# Autodesk Inventor assembly: ASY PNS 1600 Filter column D1000
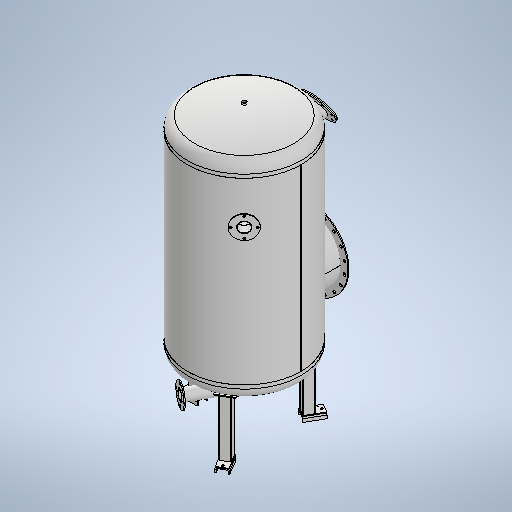
[picture p0: Inventor's stored thumbnail of the model, 512x512]
Saved by Autodesk Inventor 2025.3 (Build 293356030, 356C)
## iProperties
Created: 2025-02-13
Part Number: ASY PNS 1600 Filter column D1000
Document SubType Name: Assembly
Designer: pokla
Author: pokla
Revision Number: 3
## Documents named in this file (23)
- C:\Users\admin\Yandex.Disk\home pc\Inventor\SLM Salemal\ASY SLM 1600 Filter column D1000.iam
- C:\Users\admin\Yandex.Disk\home pc\Inventor\SLM Salemal\PNS-612 accses hatch flangeipt.ipt
- C:\Users\admin\Yandex.Disk\home pc\Inventor\SLM Salemal\PNS 1601 DIM Filter column D1000.ipt
- C:\Users\admin\Yandex.Disk\home pc\Inventor\SLM Salemal\PNS-611 accses hatch tube.ipt
- C:\Users\admin\Yandex.Disk\home pc\Inventor\SLM Salemal\PNS 1602 main Shell D1000.ipt
- C:\Users\admin\Yandex.Disk\home pc\Inventor\SLM Salemal\PNS 1604 dished head D1000.ipt
- C:\Users\admin\Yandex.Disk\home pc\Inventor\SLM Salemal\Fitting G1.ipt
- C:\Users\admin\Yandex.Disk\home pc\Inventor\SLM Salemal\ASY PNS 1690 Filter legs D1000.iam
- C:\Users\admin\Yandex.Disk\home pc\Inventor\SLM Salemal\PNS 1633 charging blind flange.ipt
- C:\Users\admin\Yandex.Disk\home pc\Inventor\SLM Salemal\ASY PNS 1610 charging hatch.iam
- C:\Users\admin\Yandex.Disk\home pc\Inventor\Content Center Files\en-US\JIS B 2312 90 (2)\JIS B 2312 90 Deg Long Elbow Steel 80A x Sch 40.ipt
- C:\Users\admin\Yandex.Disk\home pc\Inventor\SLM Salemal\ASY PNS 1650 filter-distribution-system 1000.iam
- C:\Users\admin\Yandex.Disk\home pc\Inventor\SLM Salemal\PNS 1612 FDS tube 2.ipt
- C:\Users\admin\Yandex.Disk\home pc\Inventor\SLM Salemal\PNS 1604 charging tube.ipt
- C:\Users\admin\Yandex.Disk\home pc\Inventor\SLM Salemal\PNS 1606 charging flange round.ipt
- C:\Users\admin\Yandex.Disk\home pc\Inventor\SLM Salemal\PNS 1607 charging flange cup.ipt
- C:\Users\admin\Yandex.Disk\home pc\Inventor\SLM Salemal\PNS 1613 FDS tube 3.ipt
- C:\Users\admin\Yandex.Disk\home pc\Inventor\SLM Salemal\PNS 1614 FDS tube 4.ipt
- C:\Users\admin\Yandex.Disk\home pc\Inventor\SLM Salemal\PNS 1615 FDS tube 5.ipt
- C:\Users\admin\Yandex.Disk\home pc\Inventor\SLM Salemal\ASY PNS 179 top funnel 1200 50-90_1000x90.iam
- C:\Users\admin\Yandex.Disk\home pc\Inventor\SLM Salemal\pallet jack dummy.ipt
- C:\Users\admin\Yandex.Disk\home pc\Inventor\SLM Salemal\SLM 1431 FDS flange DN90.ipt
- C:\Users\admin\Yandex.Disk\home pc\Inventor\SLM Salemal\SLM 1432 FDS free flange DN90.ipt
## Components (27 placed, 23 different names)
1. PNS 1601 DIM Filter column D1000.ipt:1
2. PNS-612 accses hatch flangeipt.ipt:1 — Rotational:73, Rotational:74
3. PNS-611 accses hatch tube.ipt:1 — Rigid:10, Rotational:74
4. PNS 1602 main Shell D1000.ipt:1 — Rigid:10, Rigid:13, Rigid:14, Mate:1, Mate:2, Rigid:66, Rigid:74
5. PNS 1604 dished head D1000.ipt:1 — Rigid:13, Rigid:75
6. PNS 1604 dished head D1000.ipt:2 — Rigid:14, Rigid:15, Mate:3
7. Fitting G1.ipt:1 — Rigid:15
8. Fitting G1.ipt:2
9. ASY PNS 1690 Filter legs D1000.iam:1 [sub-assembly] — Flush:2, Flush:3
10. ASY PNS 1610 charging hatch.iam:1 [sub-assembly] — Rotational:73
11. PNS 1633 charging blind flange.ipt:2 — Rigid:67
12. JIS B 2312 90 Deg Long Elbow Steel 80A x Sch 40.ipt:1 — Rigid:68, Rotational:70
13. JIS B 2312 90 Deg Long Elbow Steel 80A x Sch 40.ipt:2 — Rigid:62, Rigid:73
14. ASY PNS 1650 filter-distribution-system 1000.iam:1 [sub-assembly]
15. PNS 1612 FDS tube 2:3 — Rigid:62, Rigid:78
16. PNS 1604 charging tube:1 — Rigid:64, Rigid:66
17. PNS 1606 charging flange round:1 — Rigid:64, Rigid:65
18. PNS 1607 charging flange cup:1 — Rigid:65
19. PNS 1613 FDS tube 3:1 — Rigid:67, Rigid:68, Flush:3
20. PNS 1614 FDS tube 4:1 — Rotational:70, Rigid:75, Rotational:71
21. PNS 1615 FDS tube 5:1 — Rigid:73, Rigid:74, Rigid:77
22. ASY PNS 179 top funnel 1200 50-90_1000x90:1 [sub-assembly] — Rotational:72
23. pallet jack dummy:1
24. SLM 1431 FDS flange DN90:1 — Rigid:76
25. SLM 1432 FDS free flange DN90:1 — Rotational:71, Rigid:76
26. PNS 1633 charging blind flange:5 — Rigid:77
27. PNS 1633 charging blind flange:6 — Rigid:78, Rotational:72
## Relationships (26: WeldJoint 16, RevoluteJoint 5, Mate 3, Flush 2)
- Rigid:10 [WeldJoint] (66 mm): PNS-611 accses hatch tube.ipt:1 ↔ PNS 1602 main Shell D1000.ipt:1
- Rigid:13 [WeldJoint]: PNS 1602 main Shell D1000.ipt:1 ↔ PNS 1604 dished head D1000.ipt:1
- Rigid:14 [WeldJoint]: PNS 1602 main Shell D1000.ipt:1 ↔ PNS 1604 dished head D1000.ipt:2
- Rigid:15 [WeldJoint]: PNS 1604 dished head D1000.ipt:2 ↔ Fitting G1.ipt:1
- Mate:1: PNS 1602 main Shell D1000.ipt:1
- Mate:2: PNS 1602 main Shell D1000.ipt:1
- Mate:3 (2300 mm): PNS 1604 dished head D1000.ipt:2
- Flush:2: ASY PNS 1690 Filter legs D1000.iam:1
- Rigid:62 [WeldJoint]: JIS B 2312 90 Deg Long Elbow Steel 80A x Sch 40.ipt:2 ↔ PNS 1612 FDS tube 2:3
- Rigid:64 [WeldJoint]: PNS 1604 charging tube:1 ↔ PNS 1606 charging flange round:1
- Rigid:65 [WeldJoint]: PNS 1606 charging flange round:1 ↔ PNS 1607 charging flange cup:1
- Rigid:66 [WeldJoint]: PNS 1602 main Shell D1000.ipt:1 ↔ PNS 1604 charging tube:1
- Rigid:67 [WeldJoint]: PNS 1633 charging blind flange.ipt:2 ↔ PNS 1613 FDS tube 3:1
- Rigid:68 [WeldJoint]: JIS B 2312 90 Deg Long Elbow Steel 80A x Sch 40.ipt:1 ↔ PNS 1613 FDS tube 3:1
- Rotational:70 [RevoluteJoint]: JIS B 2312 90 Deg Long Elbow Steel 80A x Sch 40.ipt:1 ↔ PNS 1614 FDS tube 4:1
- Rigid:73 [WeldJoint]: JIS B 2312 90 Deg Long Elbow Steel 80A x Sch 40.ipt:2 ↔ PNS 1615 FDS tube 5:1
- Rigid:74 [WeldJoint] (80 mm): PNS 1602 main Shell D1000.ipt:1 ↔ PNS 1615 FDS tube 5:1
- Rigid:75 [WeldJoint] (-50 mm): PNS 1604 dished head D1000.ipt:1 ↔ PNS 1614 FDS tube 4:1
- Flush:3: ASY PNS 1690 Filter legs D1000.iam:1 ↔ PNS 1613 FDS tube 3:1
- Rotational:71 [RevoluteJoint]: PNS 1614 FDS tube 4:1 ↔ SLM 1432 FDS free flange DN90:1
- Rigid:76 [WeldJoint]: SLM 1431 FDS flange DN90:1 ↔ SLM 1432 FDS free flange DN90:1
- Rigid:77 [WeldJoint]: PNS 1615 FDS tube 5:1 ↔ PNS 1633 charging blind flange:5
- Rigid:78 [WeldJoint]: PNS 1612 FDS tube 2:3 ↔ PNS 1633 charging blind flange:6
- Rotational:72 [RevoluteJoint]: ASY PNS 179 top funnel 1200 50-90_1000x90:1 ↔ PNS 1633 charging blind flange:6
- Rotational:73 [RevoluteJoint]: PNS-612 accses hatch flangeipt.ipt:1 ↔ ASY PNS 1610 charging hatch.iam:1
- Rotational:74 [RevoluteJoint]: PNS-612 accses hatch flangeipt.ipt:1 ↔ PNS-611 accses hatch tube.ipt:1
